# Autodesk Inventor assembly: rotor
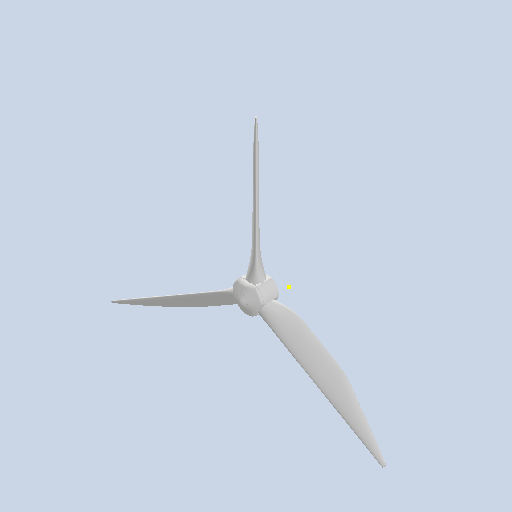
[picture p0: Inventor's stored thumbnail of the model, 512x512]
Saved by Autodesk Inventor 2023 (Build 270158000, 158)
## iProperties
Created: 2023-09-18
Part Number: rotor
Document SubType Name: Assembly
Designer: alexa
Author: alexa
## Documents named in this file (5)
- C:\Users\alexa\OneDrive - Stredni prumyslova skola\Desktop\Inventor\Vetrna elektrarna\rotor.iam
- C:\Users\alexa\OneDrive - Stredni prumyslova skola\Desktop\Inventor\Vetrna elektrarna\VickoNaSpojkuBlejdu.ipt
- C:\Users\alexa\OneDrive - Stredni prumyslova skola\Desktop\Inventor\Vetrna elektrarna\SpojkaBlejdu.ipt
- C:\Users\alexa\OneDrive - Stredni prumyslova skola\Desktop\Inventor\Vetrna elektrarna\Blejd.ipt
- C:\Users\alexa\OneDrive - Stredni prumyslova skola\Desktop\Inventor\Vetrna elektrarna\Nos.ipt
## Components (6 placed, 4 different names)
1. VickoNaSpojkuBlejdu:1 — Mate:8, Mate:9, Mate:10, Mate:11, Mate:12
2. SpojkaBlejdu:1 — Mate:1, Mate:2, Mate:3, Mate:4, Mate:5, Mate:6, Mate:7, Mate:8, Mate:9, Mate:10
3. Blejd:1 — Mate:6, Mate:7
4. Blejd:2 — Mate:4, Mate:5
5. Blejd:3 — Mate:1, Mate:2, Mate:3
6. Nos:1 — Mate:11, Mate:12
## Relationships (12: Mate 12)
- Mate:1: SpojkaBlejdu:1 ↔ Blejd:3
- Mate:2: SpojkaBlejdu:1 ↔ Blejd:3
- Mate:3: SpojkaBlejdu:1 ↔ Blejd:3
- Mate:4: SpojkaBlejdu:1 ↔ Blejd:2
- Mate:5: SpojkaBlejdu:1 ↔ Blejd:2
- Mate:6: SpojkaBlejdu:1 ↔ Blejd:1
- Mate:7: SpojkaBlejdu:1 ↔ Blejd:1
- Mate:8: VickoNaSpojkuBlejdu:1 ↔ SpojkaBlejdu:1
- Mate:9: VickoNaSpojkuBlejdu:1 ↔ SpojkaBlejdu:1
- Mate:10: VickoNaSpojkuBlejdu:1 ↔ SpojkaBlejdu:1
- Mate:11: VickoNaSpojkuBlejdu:1 ↔ Nos:1
- Mate:12: VickoNaSpojkuBlejdu:1 ↔ Nos:1
